# Autodesk Inventor assembly: 6P Sprocket
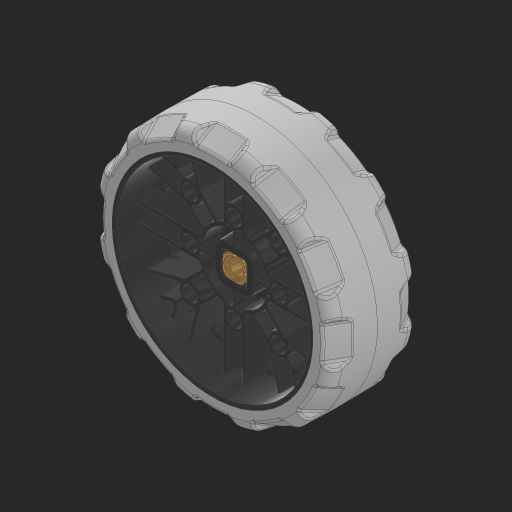
[picture p0: Inventor's stored thumbnail of the model, 512x512]
Saved by Autodesk Inventor 2023 (Build 270158000, 158)
## iProperties
Created: 2022-08-02
Part Number: 6P Sprocket
Document SubType Name: Assembly
Designer: ylu12
Author: ylu12
## Documents named in this file (4)
- C:\Users\ylu12\Documents\GitHub\VEX-CAD-Inventor\Motion\Wheels\Traction Wheel\2.75 Traction AS, Circle.iam
- C:\Users\ylu12\Documents\GitHub\VEX-CAD-Inventor\Motion\Wheels\Reference Files\2.75 Traction Antistatic.ipt
- C:\Users\ylu12\Documents\GitHub\VEX-CAD-Inventor\Motion\HS Shaft Adapter Circle.ipt
- C:\Users\ylu12\Documents\GitHub\VEX-CAD-Inventor\Motion\Wheels\Traction Wheel.iam
## Components (2 placed, 2 different names)
1. 2.75 Traction Antistatic:1 — Mate:17, Mate:18, Mate:19
2. Circle — Mate:32, Mate:33, Flush:10
## Relationships (6: Mate 5, Flush 1)
- Mate:17: 2.75 Traction Antistatic:1
- Mate:18: 2.75 Traction Antistatic:1
- Mate:19: 2.75 Traction Antistatic:1
- Mate:32: Circle
- Mate:33: Circle
- Flush:10 (6.35 mm): Circle
## Named parameters: Thickness = 8.255 mm
